# Autodesk Inventor assembly: FullSkirt
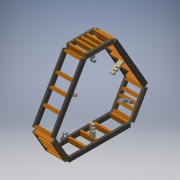
[picture p0: Inventor's stored thumbnail of the model, 180x180]
Saved by Autodesk Inventor 2016 (Build 200138000, 138)
## iProperties
Created: 2016-06-15
Part Number: FullSkirt
Document SubType Name: Assembly
Designer: cutrones
Author: cutrones
## Documents named in this file (5)
- C:\Users\cutrones\Desktop\MotionBase\CAD\MotionBaseCAD\BaseSkirt\FullSkirt.iam
- C:\Users\cutrones\Desktop\MotionBase\CAD\MotionBaseCAD\BaseSkirt\LargeSkirtWall.iam
- C:\Users\cutrones\Desktop\MotionBase\CAD\MotionBaseCAD\BaseSkirt\SmallSkirtWall.iam
- C:\Users\cutrones\Desktop\MotionBase\CAD\MotionBaseCAD\BaseSkirt\LargeSideHook.ipt
- C:\Users\cutrones\Desktop\MotionBase\CAD\MotionBaseCAD\BaseSkirt\SmallSideHook.ipt
## Components (12 placed, 4 different names)
1. LargeSkirtWall:1 [sub-assembly] — Mate:5, Flush:4, Flush:5, Mate:7, Angle:2, Mate:8, Mate:9, Mate:13, Flush:12, Flush:15
2. LargeSkirtWall:2 [sub-assembly] — Mate:2, Mate:3, Flush:3, Flush:6, Angle:1, Mate:11, Flush:10, Flush:13
3. LargeSkirtWall:3 [sub-assembly] — Mate:1, Mate:6, Flush:1, Flush:2, Angle:3, Mate:14, Flush:8, Flush:17
4. SmallSkirtWall:1 [sub-assembly] — Mate:3, Flush:5, Flush:6, Mate:7, Angle:3, Mate:12, Flush:11, Flush:14
5. SmallSkirtWall:2 [sub-assembly] — Mate:5, Mate:6, Flush:1, Flush:4, Angle:1, Mate:15, Flush:7, Flush:16
6. SmallSkirtWall:3 [sub-assembly] — Mate:1, Mate:2, Flush:2, Flush:3, Angle:2, Mate:10, Flush:9, Flush:18
7. LargeSideHook:1 — Mate:11, Flush:10, Flush:13
8. LargeSideHook:2 — Mate:14, Flush:8, Flush:17
9. LargeSideHook:3 — Mate:13, Flush:12, Flush:15
10. SmallSideHook:1 — Mate:10, Flush:9, Flush:18
11. SmallSideHook:2 — Mate:15, Flush:7, Flush:16
12. SmallSideHook:3 — Mate:12, Flush:11, Flush:14
## Relationships (35: Flush 18, Mate 14, Angle 3)
- Mate:1: LargeSkirtWall:3 ↔ SmallSkirtWall:3
- Mate:2: LargeSkirtWall:2 ↔ SmallSkirtWall:3
- Mate:3: LargeSkirtWall:2 ↔ SmallSkirtWall:1
- Mate:5: LargeSkirtWall:1 ↔ SmallSkirtWall:2
- Mate:6: LargeSkirtWall:3 ↔ SmallSkirtWall:2
- Flush:1: LargeSkirtWall:3 ↔ SmallSkirtWall:2
- Flush:2: LargeSkirtWall:3 ↔ SmallSkirtWall:3
- Flush:3: LargeSkirtWall:2 ↔ SmallSkirtWall:3
- Flush:4: LargeSkirtWall:1 ↔ SmallSkirtWall:2
- Flush:5: LargeSkirtWall:1 ↔ SmallSkirtWall:1
- Flush:6: LargeSkirtWall:2 ↔ SmallSkirtWall:1
- Mate:7: LargeSkirtWall:1 ↔ SmallSkirtWall:1
- Angle:1 (0 deg): LargeSkirtWall:2 ↔ SmallSkirtWall:2
- Angle:2 (180 deg): LargeSkirtWall:1 ↔ SmallSkirtWall:3
- Angle:3 (180 deg): LargeSkirtWall:3 ↔ SmallSkirtWall:1
- Mate:8: LargeSkirtWall:1
- Mate:9: LargeSkirtWall:1
- Mate:10: SmallSkirtWall:3 ↔ SmallSideHook:1
- Mate:11: LargeSkirtWall:2 ↔ LargeSideHook:1
- Mate:12: SmallSkirtWall:1 ↔ SmallSideHook:3
- Mate:13: LargeSkirtWall:1 ↔ LargeSideHook:3
- Mate:14: LargeSkirtWall:3 ↔ LargeSideHook:2
- Mate:15: SmallSkirtWall:2 ↔ SmallSideHook:2
- Flush:7: SmallSkirtWall:2 ↔ SmallSideHook:2
- Flush:8: LargeSkirtWall:3 ↔ LargeSideHook:2
- Flush:9: SmallSkirtWall:3 ↔ SmallSideHook:1
- Flush:10: LargeSkirtWall:2 ↔ LargeSideHook:1
- Flush:11: SmallSkirtWall:1 ↔ SmallSideHook:3
- Flush:12: LargeSkirtWall:1 ↔ LargeSideHook:3
- Flush:13 (107.95 mm): LargeSkirtWall:2 ↔ LargeSideHook:1
- Flush:14 (-107.95 mm): SmallSkirtWall:1 ↔ SmallSideHook:3
- Flush:15 (107.95 mm): LargeSkirtWall:1 ↔ LargeSideHook:3
- Flush:16 (107.95 mm): SmallSkirtWall:2 ↔ SmallSideHook:2
- Flush:17 (107.95 mm): LargeSkirtWall:3 ↔ LargeSideHook:2
- Flush:18 (107.95 mm): SmallSkirtWall:3 ↔ SmallSideHook:1
